# Autodesk Inventor assembly: Assembly2
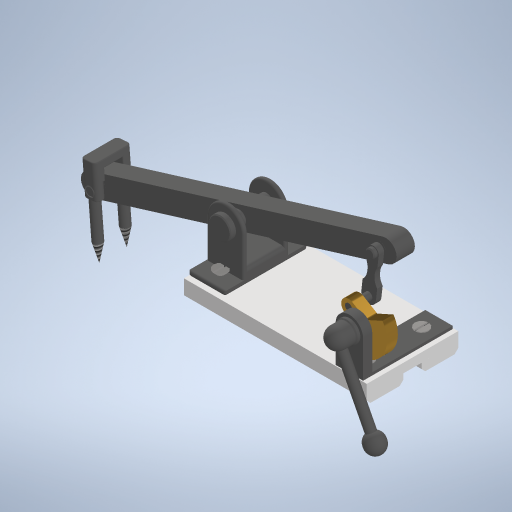
[picture p0: Inventor's stored thumbnail of the model, 512x512]
Saved by Autodesk Inventor 2024 (Build 280153000, 153)
## iProperties
Created: 2023-05-09
Part Number: Assembly2
Document SubType Name: Assembly
Designer: Raj
Author: Raj
## Documents named in this file (15)
- D:\New folder\assembly\assembly\Assembly.iam
- Assembly1.iam
- D:\New folder\assembly\Groundplate.ipt
- D:\New folder\assembly\Rail stand.ipt
- D:\New folder\assembly\Half Bearing Block.ipt
- D:\New folder\assembly\short bolt.ipt
- D:\New folder\assembly\KURBEL PART 8.ipt
- D:\New folder\assembly\PLEUEL short new.ipt
- D:\New folder\assembly\Bearing Block.ipt
- D:\New folder\assembly\Lever.ipt
- D:\New folder\assembly\Lock pin.ipt
- D:\New folder\assembly\Bolt.ipt
- C:\Users\USER\OneDrive\Documents\Inventor\Content Center Files\R2024\en-US\DIN 963\DIN 963 - M4 x 12.ipt
- D:\New folder\assembly\KURBELZAPFEN NEW.ipt
- D:\New folder\assembly\Pin Marker.ipt
## Components (18 placed, 13 different names)
1. Groundplate:1 — Mate:1, Flush:1, Flush:2, Mate:2, Flush:3, Flush:4, Mate:3, Mate:4, Mate:5, Mate:12, Mate:13, Mate:14, Insert:25, Insert:26
2. Rail stand:1 — Mate:1, Flush:1, Flush:2
3. Rail stand:2 — Mate:2, Flush:3, Flush:4
4. Half Bearing Block:2 — Mate:3, Mate:4, Mate:5, Mate:10, Mate:11, Mate:27, Mate:29
5. short bolt:1 — Mate:10, Mate:11, Mate:27, Mate:28, Flush:5, Rotation:25
6. PLEUEL short new:2 — Mate:16, Mate:17, Mate:31, Flush:7
7. Bearing Block:1 — Mate:12, Mate:13, Mate:14, Insert:1, Insert:27, Mate:32, Mate:33
8. Lever:1 — Mate:20, Mate:34, Flush:8, Mate:35, Flush:9
9. Lock pin:1 — Mate:16, Mate:17, Mate:20, Flush:8
10. Bolt:1 — Mate:32, Mate:33, Mate:34
11. DIN 963 - replaced by DIN EN ISO 2009 M4 x 12:1 — Insert:1
12. DIN 963 - replaced by DIN EN ISO 2009 M4 x 12:2 — Insert:27
13. DIN 963 - replaced by DIN EN ISO 2009 M4 x 12:3 — Insert:26
14. DIN 963 - replaced by DIN EN ISO 2009 M4 x 12:4 — Insert:25
15. KURBEL PART 8:1 — Mate:28, Mate:29, Flush:5, Rotation:25, Mate:30, Flush:6
16. KURBELZAPFEN NEW:1 — Mate:30, Flush:6, Mate:31, Flush:7
17. Pin Marker:1 — Mate:36, Flush:10
18. Lock pin:2 — Mate:35, Flush:9, Mate:36, Flush:10
## Relationships (38: Mate 23, Flush 10, Insert 4, RelateRotation 1)
- Mate:1: Groundplate:1 ↔ Rail stand:1
- Flush:1: Groundplate:1 ↔ Rail stand:1
- Flush:2: Groundplate:1 ↔ Rail stand:1
- Mate:2: Groundplate:1 ↔ Rail stand:2
- Flush:3: Groundplate:1 ↔ Rail stand:2
- Flush:4: Groundplate:1 ↔ Rail stand:2
- Mate:3: Groundplate:1 ↔ Half Bearing Block:2
- Mate:4: Groundplate:1 ↔ Half Bearing Block:2
- Mate:5: Groundplate:1 ↔ Half Bearing Block:2
- Mate:10: Half Bearing Block:2 ↔ short bolt:1
- Mate:11: Half Bearing Block:2 ↔ short bolt:1
- Mate:27: Half Bearing Block:2 ↔ short bolt:1
- Mate:12: Groundplate:1 ↔ Bearing Block:1
- Mate:13: Groundplate:1 ↔ Bearing Block:1
- Mate:14: Groundplate:1 ↔ Bearing Block:1
- Mate:16: PLEUEL short new:2 ↔ Lock pin:1
- Mate:17: PLEUEL short new:2 ↔ Lock pin:1
- Mate:20: Lever:1 ↔ Lock pin:1
- Insert:1: Bearing Block:1 ↔ DIN 963 - replaced by DIN EN ISO 2009 M4 x 12:1
- Insert:25: Groundplate:1 ↔ DIN 963 - replaced by DIN EN ISO 2009 M4 x 12:4
- Insert:26: Groundplate:1 ↔ DIN 963 - replaced by DIN EN ISO 2009 M4 x 12:3
- Insert:27: Bearing Block:1 ↔ DIN 963 - replaced by DIN EN ISO 2009 M4 x 12:2
- Mate:28: short bolt:1 ↔ KURBEL PART 8:1
- Mate:29: Half Bearing Block:2 ↔ KURBEL PART 8:1
- Flush:5: short bolt:1 ↔ KURBEL PART 8:1
- Rotation:25 [RelateRotation] (1 ul): short bolt:1 ↔ KURBEL PART 8:1
- Mate:30: KURBEL PART 8:1 ↔ KURBELZAPFEN NEW:1
- Flush:6: KURBEL PART 8:1 ↔ KURBELZAPFEN NEW:1
- Mate:31: PLEUEL short new:2 ↔ KURBELZAPFEN NEW:1
- Flush:7: PLEUEL short new:2 ↔ KURBELZAPFEN NEW:1
- Mate:32: Bearing Block:1 ↔ Bolt:1
- Mate:33: Bearing Block:1 ↔ Bolt:1
- Mate:34: Lever:1 ↔ Bolt:1
- Flush:8: Lever:1 ↔ Lock pin:1
- Mate:35: Lever:1 ↔ Lock pin:2
- Flush:9: Lever:1 ↔ Lock pin:2
- Mate:36: Pin Marker:1 ↔ Lock pin:2
- Flush:10: Pin Marker:1 ↔ Lock pin:2
